# Autodesk Inventor assembly: speaker_assembly_v2
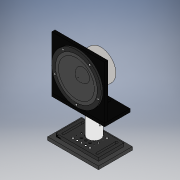
[picture p0: Inventor's stored thumbnail of the model, 180x180]
Saved by Autodesk Inventor 2019 (Build 230136000, 136)
## iProperties
Created: 2019-03-08
Part Number: speaker_assembly_v2
Document SubType Name: Assembly
Designer: Wilson Lab
Author: Wilson Lab
## Documents named in this file (8)
- C:\code\auditory-behavior-experiments\design-files\speaker-assembly\speaker_assembly_v2.iam
- C:\code\auditory-behavior-experiments\design-files\speaker-mount\speaker_mount_face.ipt
- C:\code\auditory-behavior-experiments\design-files\speaker-mount\speaker_mount_base.ipt
- C:\code\auditory-behavior-experiments\design-files\speaker-assembly\BA2-Solidworks.ipt
- C:\code\auditory-behavior-experiments\design-files\speaker-assembly\BA4-Solidworks.ipt
- C:\code\auditory-behavior-experiments\design-files\speaker-assembly\P3-Solidworks.ipt
- C:\code\auditory-behavior-experiments\design-files\speaker\8530K01_speaker.ipt
- C:\code\auditory-behavior-experiments\design-files\speaker-assembly\speaker-base-sorbothane.ipt
## Components (7 placed, 7 different names)
1. speaker_mount_face:1 — Flush:1, Mate:1, Flush:2, Mate:4, Rotational:2
2. speaker_mount_base:1 — Flush:1, Mate:1, Flush:2, Rigid:2
3. BA2-Solidworks:1 — Rotational:1, Rigid:2
4. BA4-Solidworks:1 — Rigid:1, Flush:3, Flush:4
5. P3-Solidworks:1 — Rigid:1, Rotational:1
6. 8530K01_speaker:1 — Mate:4, Rotational:2
7. speaker-base-sorbothane:1 — Flush:3, Flush:4
## Relationships (10: Flush 4, Mate 2, WeldJoint 2, RevoluteJoint 2)
- Flush:1: speaker_mount_face:1 ↔ speaker_mount_base:1
- Mate:1: speaker_mount_face:1 ↔ speaker_mount_base:1
- Flush:2: speaker_mount_face:1 ↔ speaker_mount_base:1
- Mate:4: speaker_mount_face:1 ↔ 8530K01_speaker:1
- Rigid:1 [WeldJoint]: BA4-Solidworks:1 ↔ P3-Solidworks:1
- Rotational:1 [RevoluteJoint]: BA2-Solidworks:1 ↔ P3-Solidworks:1
- Rigid:2 [WeldJoint]: speaker_mount_base:1 ↔ BA2-Solidworks:1
- Rotational:2 [RevoluteJoint]: speaker_mount_face:1 ↔ 8530K01_speaker:1
- Flush:3: BA4-Solidworks:1 ↔ speaker-base-sorbothane:1
- Flush:4: BA4-Solidworks:1 ↔ speaker-base-sorbothane:1
